# Autodesk Inventor assembly: SHOT_1_002_ShooterAssembly
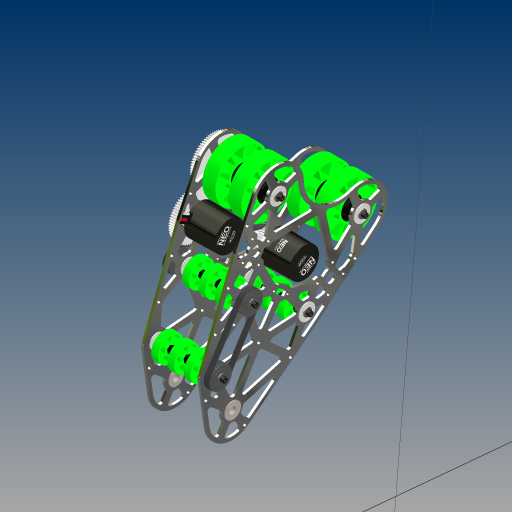
[picture p0: Inventor's stored thumbnail of the model, 512x512]
Saved by Autodesk Inventor 2024.3 (Build 283343000, 343)
## iProperties
Created: 2024-08-07
Part Number: SHOT_1_002_ShooterAssembly
Document SubType Name: Assembly
Designer: Kenji
Mass: 1474.99 g
Surface Area: 3908.93 cm^2
Volume: 710.058 cm^3
Density: 2.07728 g/cm^3
Author: Kenji
## Documents named in this file (27)
- C:\Users\Kenji\Documents\GitHub\1622-2024-Summer-CAD-A-Thon\Shooter\SHOT_1_002_ShooterAssembly.iam
- C:\Users\Kenji\Documents\GitHub\1622-2024-Summer-CAD-A-Thon\Shooter\SHOT_1_001_ShooterPlate.ipt
- C:\Users\Kenji\Documents\GitHub\1622-2024-Summer-CAD-A-Thon\COTS Library\Motion\Wheels\Compliant Wheels\4in compliant wheels\0.500in hex bore\COTS_am-3462_4indiameter_0.500inhexbore_durometer35A_CompliantWheel.ipt
- C:\Users\Kenji\Documents\GitHub\1622-2024-Summer-CAD-A-Thon\COTS Library\Motion\Bearings\COTS_WCP-0783_1.125ODHexBearing.ipt
- C:\Users\Kenji\Documents\GitHub\1622-2024-Summer-CAD-A-Thon\COTS Library\Motion\Bearings\COTS_WCP-0781_0.5ODCircularFlangedBearing.ipt
- C:\Users\Kenji\Documents\GitHub\1622-2024-Summer-CAD-A-Thon\COTS Library\Motors\COTS_REV-21-1650-V1.1_Neo1.1.ipt
- C:\Users\Kenji\Documents\GitHub\1622-2024-Summer-CAD-A-Thon\COTS Library\Motion\Wheels\Compliant Wheels\2in compliant wheels\0.500in hex bore\COTS_am-3462_2indiameter_0.500inhexbore_durometer35A_CompliantWheel.ipt
- C:\Users\Kenji\Documents\GitHub\1622-2024-Summer-CAD-A-Thon\COTS Library\Fasteners\Bolts\Button-Head\10-32\COTS_92949A265_1-2in long Stainless Steel Button Head Screw.ipt
- C:\Users\Kenji\Documents\GitHub\1622-2024-Summer-CAD-A-Thon\COTS Library\Motion\Pulleys\HTD5M\10mm Wide\COTS_HTD5M10mm24T_WCP-0564.ipt
- C:\Users\Kenji\Documents\GitHub\1622-2024-Summer-CAD-A-Thon\COTS Library\Adapters\COTS_REV-21-1879_8mmKeyTo0.5Hex.ipt
- C:\Users\Kenji\Documents\GitHub\1622-2024-Summer-CAD-A-Thon\COTS Library\Motion\Gears\20DP gears\Aluminum\COTS_WCP-0171_66T.ipt
- C:\Users\Kenji\Documents\GitHub\1622-2024-Summer-CAD-A-Thon\Shooter\SHOT_1_004_66TGear-24TPulley.ipt
- C:\Users\Kenji\Documents\GitHub\1622-2024-Summer-CAD-A-Thon\COTS Library\Motion\Gears\20DP gears\Aluminum\COTS_WCP-0717_54T.ipt
- C:\Users\Kenji\Documents\GitHub\1622-2024-Summer-CAD-A-Thon\Shooter\SHOT_1_005_36TGear-24TPulley.ipt
- C:\Users\Kenji\Documents\GitHub\1622-2024-Summer-CAD-A-Thon\Shooter\SHOT_1_014_Belt3.ipt
- C:\Users\Kenji\Documents\GitHub\1622-2024-Summer-CAD-A-Thon\Shooter\SHOT_1_013_Belt2.ipt
- C:\Users\Kenji\Documents\GitHub\1622-2024-Summer-CAD-A-Thon\Shooter\SHOT_1_012_Belt1.ipt
- C:\Users\Kenji\Documents\GitHub\1622-2024-Summer-CAD-A-Thon\Shooter\SHOT_1_010_Spacer1.ipt
- C:\Users\Kenji\Documents\GitHub\1622-2024-Summer-CAD-A-Thon\Shooter\SHOT_1_011_Spacer2.ipt
- C:\Users\Kenji\Documents\GitHub\1622-2024-Summer-CAD-A-Thon\Shooter\SHOT_1_006_HexShaft1.ipt
- C:\Users\Kenji\Documents\GitHub\1622-2024-Summer-CAD-A-Thon\Shooter\SHOT_1_007_HexShaft2.ipt
- C:\Users\Kenji\Documents\GitHub\1622-2024-Summer-CAD-A-Thon\Shooter\SHOT_1_008_HexShaft3.ipt
- C:\Users\Kenji\Documents\GitHub\1622-2024-Summer-CAD-A-Thon\Shooter\SHOT_1_009_HexShaft4.ipt
- C:\Users\Kenji\Documents\GitHub\1622-2024-Summer-CAD-A-Thon\COTS Library\Fasteners\Bolts\Socket-Head\0.25-20\COTS_91251A539_Black-Oxide Alloy Steel Socket Head Screw (1).ipt
- C:\Users\Kenji\Documents\GitHub\1622-2024-Summer-CAD-A-Thon\COTS Library\Fasteners\Washers\COTS_90107A029_316 Stainless Steel Washer.ipt
- C:\Users\Kenji\Documents\GitHub\1622-2024-Summer-CAD-A-Thon\COTS Library\Fasteners\Bolts\Button-Head\10-32\COTS_92949A267_18-8 Stainless Steel Button Head Hex Drive Screw (1).ipt
- C:\Users\Kenji\Documents\GitHub\1622-2024-Summer-CAD-A-Thon\COTS Library\Fasteners\Washers\COTS_91860A047_Size10Washer.ipt
## Components (85 placed, 26 different names)
1. SHOT_1_001_ShooterPlate:1 — Mate:140, Mate:141, Mate:142, Mate:143, Mate:144, Mate:148, Mate:150, Mate:151, Mate:152, Mate:160, Mate:161, Mate:163, Mate:164, Mate:165, Mate:166, Mate:167, Mate:168, Mate:169, Mate:170, Mate:171, Mate:172, Mate:270, Mate:271, Mate:280, Mate:281, Mate:282, Mate:283, Mate:284, Mate:285, Mate:286, Mate:287, Mate:288, Mate:289, Mate:290, Mate:294, Mate:304, Mate:305
2. SHOT_1_001_ShooterPlate:2 — Mate:140, Mate:141, Mate:147, Mate:149, Mate:156, Mate:158, Mate:159, Mate:272, Mate:273, Mate:304, Mate:311
3. COTS_WCP-0783_1.125ODHexBearing:1 — Mate:139, Flush:5, Mate:156, Mate:246
4. COTS_WCP-0783_1.125ODHexBearing:2 — Mate:146, Mate:147, Mate:149, Mate:299
5. COTS_WCP-0783_1.125ODHexBearing:3 — Mate:36, Mate:102, Flush:5, Mate:251
6. COTS_WCP-0783_1.125ODHexBearing:5 — Mate:244, Mate:270, Mate:271, Mate:274, Mate:275
7. COTS_WCP-0783_1.125ODHexBearing:9 — Mate:102, Flush:4, Mate:150, Mate:152, Mate:186, Mate:187
8. COTS_WCP-0783_1.125ODHexBearing:10 — Mate:31, Mate:104, Flush:4, Mate:151, Mate:188, Mate:213
9. COTS_WCP-0783_1.125ODHexBearing:11 — Mate:49, Mate:52, Mate:143, Mate:144, Flush:17
10. COTS_WCP-0783_1.125ODHexBearing:12 — Mate:272, Mate:273, Mate:278
11. COTS_WCP-0781_0.5ODCircularFlangedBearing:1 — Mate:138, Mate:158, Mate:159
12. COTS_WCP-0781_0.5ODCircularFlangedBearing:2 — Mate:138, Mate:160
13. COTS_REV-21-1650-V1.1_Neo1.1:1 — Mate:133, Mate:161, Mate:163, Mate:185, Mate:256, Mate:260, Mate:261, Mate:266
14. COTS_92949A265_1-2in long Stainless Steel Button Head Screw:1 — Mate:165, Mate:168, Mate:185
15. COTS_92949A265_1-2in long Stainless Steel Button Head Screw:2 — Mate:167, Mate:170
16. COTS_92949A265_1-2in long Stainless Steel Button Head Screw:3 — Mate:166, Mate:169
17. COTS_92949A265_1-2in long Stainless Steel Button Head Screw:4 — Mate:164, Mate:171
18. COTS_WCP-0783_1.125ODHexBearing:13 — Mate:148, Mate:297, Mate:305, Mate:306
19. COTS_WCP-0783_1.125ODHexBearing:14 — Mate:134, Mate:308, Mate:311, Mate:315
20. COTS_REV-21-1650-V1.1_Neo1.1:2 — Mate:280, Mate:281, Mate:282, Mate:291, Mate:292, Mate:293, Mate:295
21. COTS_REV-21-1879_8mmKeyTo0.5Hex:1 — Mate:291, Mate:292
22. COTS_92949A265_1-2in long Stainless Steel Button Head Screw:5 — Mate:285, Mate:288
23. COTS_92949A265_1-2in long Stainless Steel Button Head Screw:6 — Mate:286, Mate:290
24. COTS_92949A265_1-2in long Stainless Steel Button Head Screw:7 — Mate:283, Mate:287
25. COTS_92949A265_1-2in long Stainless Steel Button Head Screw:8 — Mate:284, Mate:289
26. SHOT_1_004_66TGear-24TPulley:1 — Mate:133, Mate:172, Flush:6, Mate:198, Mate:257
27. COTS_WCP-0171_66T:1 — Mate:186, Mate:187, Mate:301, Flush:15
28. COTS_HTD5M10mm24T_WCP-0564:1 — Mate:188, Flush:6, Mate:199, Mate:200, Mate:207, Flush:9, Mate:214, Mate:240
29. COTS_WCP-0717_54T:1 — Mate:274, Mate:275, Mate:276, Flush:13, Mate:329, Mate:330
30. SHOT_1_005_36TGear-24TPulley:1 — Mate:293, Mate:294, Mate:296, Flush:16, Mate:318, Mate:319
31. COTS_HTD5M10mm24T_WCP-0564:2 — Mate:298, Flush:14, Mate:299, Mate:320, Mate:323
32. COTS_HTD5M10mm24T_WCP-0564:3 — Mate:300, Flush:16, Mate:307, Mate:317, Mate:326
33. COTS_HTD5M10mm24T_WCP-0564:4 — Mate:255, Mate:314, Mate:315, Mate:321
34. SHOT_1_014_Belt3:1 — Mate:255, Mate:320, Mate:321
35. SHOT_1_013_Belt2:1 — Mate:317, Mate:318, Mate:319
36. SHOT_1_012_Belt1:1 — Mate:198, Mate:199, Mate:200
37. SHOT_1_010_Spacer1:1 — Mate:213, Mate:214
38. SHOT_1_010_Spacer1:2 — Mate:306, Mate:307
39. SHOT_1_006_HexShaft1:1 — Mate:235, Mate:301, Flush:15, Mate:302, Mate:303
40. SHOT_1_007_HexShaft2:1 — Mate:207, Flush:9, Mate:238, Mate:245
41. SHOT_1_008_HexShaft3:1 — Mate:297, Mate:298, Flush:14, Mate:300, Mate:322, Mate:325
42. SHOT_1_009_HexShaft4:1 — Mate:237, Mate:248, Mate:308, Flush:17, Mate:310, Mate:312
43. SHOT_1_006_HexShaft1:2 — Mate:239, Mate:249, Mate:276, Flush:13, Mate:277
44. COTS_91251A539_Black-Oxide Alloy Steel Socket Head Screw (1):1 — Mate:219, Mate:233, Mate:239
45. COTS_91251A539_Black-Oxide Alloy Steel Socket Head Screw (1):2 — Mate:220, Mate:230, Mate:238
46. COTS_91251A539_Black-Oxide Alloy Steel Socket Head Screw (1):3 — Mate:222, Mate:229, Mate:249
47. COTS_91251A539_Black-Oxide Alloy Steel Socket Head Screw (1):4 — Mate:217, Mate:232, Mate:303
48. COTS_91251A539_Black-Oxide Alloy Steel Socket Head Screw (1):5 — Mate:218, Mate:234, Mate:235
49. COTS_91251A539_Black-Oxide Alloy Steel Socket Head Screw (1):6 — Mate:316, Mate:322, Mate:324
50. COTS_91251A539_Black-Oxide Alloy Steel Socket Head Screw (1):7 — Mate:224, Mate:237, Mate:309
51. COTS_91251A539_Black-Oxide Alloy Steel Socket Head Screw (1):8 — Mate:223, Mate:227, Mate:325
52. COTS_91251A539_Black-Oxide Alloy Steel Socket Head Screw (1):9 — Mate:216, Mate:248, Mate:313, Mate:314
53. COTS_91251A539_Black-Oxide Alloy Steel Socket Head Screw (1):10 — Mate:215, Mate:231, Mate:245
54. COTS_90107A029_316 Stainless Steel Washer:1 — Mate:218, Mate:234, Mate:302
55. COTS_90107A029_316 Stainless Steel Washer:2 — Mate:220, Mate:230, Mate:240
56. COTS_90107A029_316 Stainless Steel Washer:3 — Mate:316, Mate:323, Mate:324
57. COTS_90107A029_316 Stainless Steel Washer:4 — Mate:219, Mate:233, Mate:244
58. COTS_90107A029_316 Stainless Steel Washer:5 — Mate:222, Mate:229, Mate:278
59. COTS_90107A029_316 Stainless Steel Washer:6 — Mate:223, Mate:227, Mate:326
60. COTS_90107A029_316 Stainless Steel Washer:7 — Mate:224, Mate:309, Mate:310
61. COTS_90107A029_316 Stainless Steel Washer:8 — Mate:217, Mate:232, Mate:251
62. COTS_90107A029_316 Stainless Steel Washer:9 — Mate:215, Mate:231, Mate:246
63. COTS_90107A029_316 Stainless Steel Washer:10 — Mate:216, Mate:312, Mate:313
64. SHOT_1_011_Spacer2:1 — Mate:256, Mate:257, Mate:267
65. SHOT_1_011_Spacer2:2 — Mate:269, Mate:279, Mate:296
66. COTS_REV-21-1879_8mmKeyTo0.5Hex:2 — Mate:260, Mate:261
67. COTS_92949A267_18-8 Stainless Steel Button Head Hex Drive Screw (1):1 — Mate:263, Mate:265, Mate:266
68. COTS_92949A267_18-8 Stainless Steel Button Head Hex Drive Screw (1):2 — Mate:262, Mate:264, Mate:279, Mate:295
69. COTS_91860A047_Size10Washer:1 — Mate:262, Mate:264, Mate:269
70. COTS_91860A047_Size10Washer:2 — Mate:263, Mate:265, Mate:267
71. COTS_90107A029_316 Stainless Steel Washer:11 — Mate:327, Mate:328, Mate:329, Mate:330
72. COTS_91251A539_Black-Oxide Alloy Steel Socket Head Screw (1):11 — Mate:327, Mate:328
73. COTS_am-3462_4indiameter_0.500inhexbore_durometer35A_CompliantWheel:4 — Mate:36, Flush:3
74. COTS_am-3462_4indiameter_0.500inhexbore_durometer35A_CompliantWheel:1 — Mate:31, Flush:3, Mate:104
75. COTS_am-3462_4indiameter_0.500inhexbore_durometer35A_CompliantWheel:5
76. COTS_am-3462_4indiameter_0.500inhexbore_durometer35A_CompliantWheel:6 — Mate:139
77. COTS_am-3462_2indiameter_0.500inhexbore_durometer35A_CompliantWheel:2 — Mate:49, Flush:1, Mate:52
78. COTS_am-3462_2indiameter_0.500inhexbore_durometer35A_CompliantWheel:6 — Flush:2
79. COTS_am-3462_2indiameter_0.500inhexbore_durometer35A_CompliantWheel:1 — Flush:1, Flush:2
80. COTS_am-3462_2indiameter_0.500inhexbore_durometer35A_CompliantWheel:7 — Mate:142
81. COTS_am-3462_2indiameter_0.500inhexbore_durometer35A_CompliantWheel:8
82. COTS_am-3462_2indiameter_0.500inhexbore_durometer35A_CompliantWheel:9
83. COTS_am-3462_2indiameter_0.500inhexbore_durometer35A_CompliantWheel:10 — Mate:134
84. COTS_am-3462_2indiameter_0.500inhexbore_durometer35A_CompliantWheel:11 — Mate:146
85. COTS_am-3462_2indiameter_0.500inhexbore_durometer35A_CompliantWheel:12 — Mate:277
## Component patterns: (2 elements, first: COTS_am-3462_4indiameter_0.500inhexbore_durometer35A_CompliantWheel:4 + COTS_am-3462_4indiameter_0.500inhexbore_durometer35A_CompliantWheel:1), (3 elements, first: COTS_am-3462_2indiameter_0.500inhexbore_durometer35A_CompliantWheel:2 + COTS_am-3462_2indiameter_0.500inhexbore_durometer35A_CompliantWheel:6 + COTS_am-3462_2indiameter_0.500inhexbore_durometer35A_CompliantWheel:1)
## Relationships (159: Mate 147, Flush 12)
- Mate:31: COTS_WCP-0783_1.125ODHexBearing:10 ↔ COTS_am-3462_4indiameter_0.500inhexbore_durometer35A_CompliantWheel:1
- Mate:36: COTS_WCP-0783_1.125ODHexBearing:3 ↔ COTS_am-3462_4indiameter_0.500inhexbore_durometer35A_CompliantWheel:4
- Mate:49: COTS_WCP-0783_1.125ODHexBearing:11 ↔ COTS_am-3462_2indiameter_0.500inhexbore_durometer35A_CompliantWheel:2
- Flush:1: COTS_am-3462_2indiameter_0.500inhexbore_durometer35A_CompliantWheel:2 ↔ COTS_am-3462_2indiameter_0.500inhexbore_durometer35A_CompliantWheel:1
- Flush:2: COTS_am-3462_2indiameter_0.500inhexbore_durometer35A_CompliantWheel:6 ↔ COTS_am-3462_2indiameter_0.500inhexbore_durometer35A_CompliantWheel:1
- Mate:52 (12.7 mm): COTS_WCP-0783_1.125ODHexBearing:11 ↔ COTS_am-3462_2indiameter_0.500inhexbore_durometer35A_CompliantWheel:2
- Mate:102: COTS_WCP-0783_1.125ODHexBearing:3 ↔ COTS_WCP-0783_1.125ODHexBearing:9
- Flush:3: COTS_am-3462_4indiameter_0.500inhexbore_durometer35A_CompliantWheel:4 ↔ COTS_am-3462_4indiameter_0.500inhexbore_durometer35A_CompliantWheel:1
- Mate:104 (12.7 mm): COTS_WCP-0783_1.125ODHexBearing:10 ↔ COTS_am-3462_4indiameter_0.500inhexbore_durometer35A_CompliantWheel:1
- Mate:133: COTS_REV-21-1650-V1.1_Neo1.1:1 ↔ SHOT_1_004_66TGear-24TPulley:1
- Mate:134: COTS_WCP-0783_1.125ODHexBearing:14 ↔ COTS_am-3462_2indiameter_0.500inhexbore_durometer35A_CompliantWheel:10
- Mate:138: COTS_WCP-0781_0.5ODCircularFlangedBearing:1 ↔ COTS_WCP-0781_0.5ODCircularFlangedBearing:2
- Mate:139: COTS_WCP-0783_1.125ODHexBearing:1 ↔ COTS_am-3462_4indiameter_0.500inhexbore_durometer35A_CompliantWheel:6
- Flush:4: COTS_WCP-0783_1.125ODHexBearing:9 ↔ COTS_WCP-0783_1.125ODHexBearing:10
- Flush:5: COTS_WCP-0783_1.125ODHexBearing:1 ↔ COTS_WCP-0783_1.125ODHexBearing:3
- Mate:140: SHOT_1_001_ShooterPlate:1 ↔ SHOT_1_001_ShooterPlate:2
- Mate:141: SHOT_1_001_ShooterPlate:1 ↔ SHOT_1_001_ShooterPlate:2
- Mate:142: SHOT_1_001_ShooterPlate:1 ↔ COTS_am-3462_2indiameter_0.500inhexbore_durometer35A_CompliantWheel:7
- Mate:143: SHOT_1_001_ShooterPlate:1 ↔ COTS_WCP-0783_1.125ODHexBearing:11
- Mate:144: SHOT_1_001_ShooterPlate:1 ↔ COTS_WCP-0783_1.125ODHexBearing:11
- Mate:146: COTS_WCP-0783_1.125ODHexBearing:2 ↔ COTS_am-3462_2indiameter_0.500inhexbore_durometer35A_CompliantWheel:11
- Mate:147: SHOT_1_001_ShooterPlate:2 ↔ COTS_WCP-0783_1.125ODHexBearing:2
- Mate:148: SHOT_1_001_ShooterPlate:1 ↔ COTS_WCP-0783_1.125ODHexBearing:13
- Mate:149: SHOT_1_001_ShooterPlate:2 ↔ COTS_WCP-0783_1.125ODHexBearing:2
- Mate:150: SHOT_1_001_ShooterPlate:1 ↔ COTS_WCP-0783_1.125ODHexBearing:9
- Mate:151: SHOT_1_001_ShooterPlate:1 ↔ COTS_WCP-0783_1.125ODHexBearing:10
- Mate:152: SHOT_1_001_ShooterPlate:1 ↔ COTS_WCP-0783_1.125ODHexBearing:9
- Mate:156: SHOT_1_001_ShooterPlate:2 ↔ COTS_WCP-0783_1.125ODHexBearing:1
- Mate:158: SHOT_1_001_ShooterPlate:2 ↔ COTS_WCP-0781_0.5ODCircularFlangedBearing:1
- Mate:159: SHOT_1_001_ShooterPlate:2 ↔ COTS_WCP-0781_0.5ODCircularFlangedBearing:1
- Mate:160: SHOT_1_001_ShooterPlate:1 ↔ COTS_WCP-0781_0.5ODCircularFlangedBearing:2
- Mate:161: SHOT_1_001_ShooterPlate:1 ↔ COTS_REV-21-1650-V1.1_Neo1.1:1
- Mate:163: SHOT_1_001_ShooterPlate:1 ↔ COTS_REV-21-1650-V1.1_Neo1.1:1
- Mate:164: SHOT_1_001_ShooterPlate:1 ↔ COTS_92949A265_1-2in long Stainless Steel Button Head Screw:4
- Mate:165: SHOT_1_001_ShooterPlate:1 ↔ COTS_92949A265_1-2in long Stainless Steel Button Head Screw:1
- Mate:166: SHOT_1_001_ShooterPlate:1 ↔ COTS_92949A265_1-2in long Stainless Steel Button Head Screw:3
- Mate:167: SHOT_1_001_ShooterPlate:1 ↔ COTS_92949A265_1-2in long Stainless Steel Button Head Screw:2
- Mate:168: SHOT_1_001_ShooterPlate:1 ↔ COTS_92949A265_1-2in long Stainless Steel Button Head Screw:1
- Mate:169: SHOT_1_001_ShooterPlate:1 ↔ COTS_92949A265_1-2in long Stainless Steel Button Head Screw:3
- Mate:170: SHOT_1_001_ShooterPlate:1 ↔ COTS_92949A265_1-2in long Stainless Steel Button Head Screw:2
- Mate:171: SHOT_1_001_ShooterPlate:1 ↔ COTS_92949A265_1-2in long Stainless Steel Button Head Screw:4
- Mate:172: SHOT_1_001_ShooterPlate:1 ↔ SHOT_1_004_66TGear-24TPulley:1
- Mate:185: COTS_REV-21-1650-V1.1_Neo1.1:1 ↔ COTS_92949A265_1-2in long Stainless Steel Button Head Screw:1
- Mate:186: COTS_WCP-0783_1.125ODHexBearing:9 ↔ COTS_WCP-0171_66T:1
- Mate:187: COTS_WCP-0783_1.125ODHexBearing:9 ↔ COTS_WCP-0171_66T:1
- Mate:188: COTS_WCP-0783_1.125ODHexBearing:10 ↔ COTS_HTD5M10mm24T_WCP-0564:1
- Flush:6: SHOT_1_004_66TGear-24TPulley:1 ↔ COTS_HTD5M10mm24T_WCP-0564:1
- Mate:198: SHOT_1_004_66TGear-24TPulley:1 ↔ SHOT_1_012_Belt1:1
- Mate:199: COTS_HTD5M10mm24T_WCP-0564:1 ↔ SHOT_1_012_Belt1:1
- Mate:200: COTS_HTD5M10mm24T_WCP-0564:1 ↔ SHOT_1_012_Belt1:1
- Mate:207: COTS_HTD5M10mm24T_WCP-0564:1 ↔ SHOT_1_007_HexShaft2:1
- Flush:9: COTS_HTD5M10mm24T_WCP-0564:1 ↔ SHOT_1_007_HexShaft2:1
- Mate:213: COTS_WCP-0783_1.125ODHexBearing:10 ↔ SHOT_1_010_Spacer1:1
- Mate:214: COTS_HTD5M10mm24T_WCP-0564:1 ↔ SHOT_1_010_Spacer1:1
- Mate:215: COTS_91251A539_Black-Oxide Alloy Steel Socket Head Screw (1):10 ↔ COTS_90107A029_316 Stainless Steel Washer:9
- Mate:216: COTS_91251A539_Black-Oxide Alloy Steel Socket Head Screw (1):9 ↔ COTS_90107A029_316 Stainless Steel Washer:10
- Mate:217: COTS_91251A539_Black-Oxide Alloy Steel Socket Head Screw (1):4 ↔ COTS_90107A029_316 Stainless Steel Washer:8
- Mate:218: COTS_91251A539_Black-Oxide Alloy Steel Socket Head Screw (1):5 ↔ COTS_90107A029_316 Stainless Steel Washer:1
- Mate:219: COTS_91251A539_Black-Oxide Alloy Steel Socket Head Screw (1):1 ↔ COTS_90107A029_316 Stainless Steel Washer:4
- Mate:220: COTS_91251A539_Black-Oxide Alloy Steel Socket Head Screw (1):2 ↔ COTS_90107A029_316 Stainless Steel Washer:2
- Mate:222: COTS_91251A539_Black-Oxide Alloy Steel Socket Head Screw (1):3 ↔ COTS_90107A029_316 Stainless Steel Washer:5
- Mate:223: COTS_91251A539_Black-Oxide Alloy Steel Socket Head Screw (1):8 ↔ COTS_90107A029_316 Stainless Steel Washer:6
- Mate:224: COTS_91251A539_Black-Oxide Alloy Steel Socket Head Screw (1):7 ↔ COTS_90107A029_316 Stainless Steel Washer:7
- Mate:227: COTS_91251A539_Black-Oxide Alloy Steel Socket Head Screw (1):8 ↔ COTS_90107A029_316 Stainless Steel Washer:6
- Mate:229: COTS_91251A539_Black-Oxide Alloy Steel Socket Head Screw (1):3 ↔ COTS_90107A029_316 Stainless Steel Washer:5
- Mate:230: COTS_91251A539_Black-Oxide Alloy Steel Socket Head Screw (1):2 ↔ COTS_90107A029_316 Stainless Steel Washer:2
- Mate:231: COTS_91251A539_Black-Oxide Alloy Steel Socket Head Screw (1):10 ↔ COTS_90107A029_316 Stainless Steel Washer:9
- Mate:232: COTS_91251A539_Black-Oxide Alloy Steel Socket Head Screw (1):4 ↔ COTS_90107A029_316 Stainless Steel Washer:8
- Mate:233: COTS_91251A539_Black-Oxide Alloy Steel Socket Head Screw (1):1 ↔ COTS_90107A029_316 Stainless Steel Washer:4
- Mate:234: COTS_91251A539_Black-Oxide Alloy Steel Socket Head Screw (1):5 ↔ COTS_90107A029_316 Stainless Steel Washer:1
- Mate:235: SHOT_1_006_HexShaft1:1 ↔ COTS_91251A539_Black-Oxide Alloy Steel Socket Head Screw (1):5
- Mate:237: SHOT_1_009_HexShaft4:1 ↔ COTS_91251A539_Black-Oxide Alloy Steel Socket Head Screw (1):7
- Mate:238: SHOT_1_007_HexShaft2:1 ↔ COTS_91251A539_Black-Oxide Alloy Steel Socket Head Screw (1):2
- Mate:239: SHOT_1_006_HexShaft1:2 ↔ COTS_91251A539_Black-Oxide Alloy Steel Socket Head Screw (1):1
- Mate:240: COTS_HTD5M10mm24T_WCP-0564:1 ↔ COTS_90107A029_316 Stainless Steel Washer:2
- Mate:244: COTS_WCP-0783_1.125ODHexBearing:5 ↔ COTS_90107A029_316 Stainless Steel Washer:4
- Mate:245: SHOT_1_007_HexShaft2:1 ↔ COTS_91251A539_Black-Oxide Alloy Steel Socket Head Screw (1):10
- Mate:246: COTS_WCP-0783_1.125ODHexBearing:1 ↔ COTS_90107A029_316 Stainless Steel Washer:9
- Mate:248: SHOT_1_009_HexShaft4:1 ↔ COTS_91251A539_Black-Oxide Alloy Steel Socket Head Screw (1):9
- Mate:249: SHOT_1_006_HexShaft1:2 ↔ COTS_91251A539_Black-Oxide Alloy Steel Socket Head Screw (1):3
- Mate:251: COTS_WCP-0783_1.125ODHexBearing:3 ↔ COTS_90107A029_316 Stainless Steel Washer:8
- Mate:255: COTS_HTD5M10mm24T_WCP-0564:4 ↔ SHOT_1_014_Belt3:1
- Mate:256: COTS_REV-21-1650-V1.1_Neo1.1:1 ↔ SHOT_1_011_Spacer2:1
- Mate:257: SHOT_1_004_66TGear-24TPulley:1 ↔ SHOT_1_011_Spacer2:1
- Mate:260: COTS_REV-21-1650-V1.1_Neo1.1:1 ↔ COTS_REV-21-1879_8mmKeyTo0.5Hex:2
- Mate:261: COTS_REV-21-1650-V1.1_Neo1.1:1 ↔ COTS_REV-21-1879_8mmKeyTo0.5Hex:2
- Mate:262: COTS_92949A267_18-8 Stainless Steel Button Head Hex Drive Screw (1):2 ↔ COTS_91860A047_Size10Washer:1
- Mate:263: COTS_92949A267_18-8 Stainless Steel Button Head Hex Drive Screw (1):1 ↔ COTS_91860A047_Size10Washer:2
- Mate:264: COTS_92949A267_18-8 Stainless Steel Button Head Hex Drive Screw (1):2 ↔ COTS_91860A047_Size10Washer:1
- Mate:265: COTS_92949A267_18-8 Stainless Steel Button Head Hex Drive Screw (1):1 ↔ COTS_91860A047_Size10Washer:2
- Mate:266: COTS_REV-21-1650-V1.1_Neo1.1:1 ↔ COTS_92949A267_18-8 Stainless Steel Button Head Hex Drive Screw (1):1
- Mate:267: SHOT_1_011_Spacer2:1 ↔ COTS_91860A047_Size10Washer:2
- Mate:269: SHOT_1_011_Spacer2:2 ↔ COTS_91860A047_Size10Washer:1
- Mate:270: SHOT_1_001_ShooterPlate:1 ↔ COTS_WCP-0783_1.125ODHexBearing:5
- Mate:271: SHOT_1_001_ShooterPlate:1 ↔ COTS_WCP-0783_1.125ODHexBearing:5
- Mate:272: SHOT_1_001_ShooterPlate:2 ↔ COTS_WCP-0783_1.125ODHexBearing:12
- Mate:273: SHOT_1_001_ShooterPlate:2 ↔ COTS_WCP-0783_1.125ODHexBearing:12
- Mate:274: COTS_WCP-0783_1.125ODHexBearing:5 ↔ COTS_WCP-0717_54T:1
- Mate:275: COTS_WCP-0783_1.125ODHexBearing:5 ↔ COTS_WCP-0717_54T:1
- Mate:276: COTS_WCP-0717_54T:1 ↔ SHOT_1_006_HexShaft1:2
- Flush:13: COTS_WCP-0717_54T:1 ↔ SHOT_1_006_HexShaft1:2
- Mate:277: SHOT_1_006_HexShaft1:2 ↔ COTS_am-3462_2indiameter_0.500inhexbore_durometer35A_CompliantWheel:12
- Mate:278: COTS_WCP-0783_1.125ODHexBearing:12 ↔ COTS_90107A029_316 Stainless Steel Washer:5
- Mate:279: SHOT_1_011_Spacer2:2 ↔ COTS_92949A267_18-8 Stainless Steel Button Head Hex Drive Screw (1):2
- Mate:280: SHOT_1_001_ShooterPlate:1 ↔ COTS_REV-21-1650-V1.1_Neo1.1:2
- Mate:281: SHOT_1_001_ShooterPlate:1 ↔ COTS_REV-21-1650-V1.1_Neo1.1:2
- Mate:282: SHOT_1_001_ShooterPlate:1 ↔ COTS_REV-21-1650-V1.1_Neo1.1:2
- Mate:283: SHOT_1_001_ShooterPlate:1 ↔ COTS_92949A265_1-2in long Stainless Steel Button Head Screw:7
- Mate:284: SHOT_1_001_ShooterPlate:1 ↔ COTS_92949A265_1-2in long Stainless Steel Button Head Screw:8
- Mate:285: SHOT_1_001_ShooterPlate:1 ↔ COTS_92949A265_1-2in long Stainless Steel Button Head Screw:5
- Mate:286: SHOT_1_001_ShooterPlate:1 ↔ COTS_92949A265_1-2in long Stainless Steel Button Head Screw:6
- Mate:287: SHOT_1_001_ShooterPlate:1 ↔ COTS_92949A265_1-2in long Stainless Steel Button Head Screw:7
- Mate:288: SHOT_1_001_ShooterPlate:1 ↔ COTS_92949A265_1-2in long Stainless Steel Button Head Screw:5
- Mate:289: SHOT_1_001_ShooterPlate:1 ↔ COTS_92949A265_1-2in long Stainless Steel Button Head Screw:8
- Mate:290: SHOT_1_001_ShooterPlate:1 ↔ COTS_92949A265_1-2in long Stainless Steel Button Head Screw:6
- Mate:291: COTS_REV-21-1650-V1.1_Neo1.1:2 ↔ COTS_REV-21-1879_8mmKeyTo0.5Hex:1
- Mate:292: COTS_REV-21-1650-V1.1_Neo1.1:2 ↔ COTS_REV-21-1879_8mmKeyTo0.5Hex:1
- Mate:293: COTS_REV-21-1650-V1.1_Neo1.1:2 ↔ SHOT_1_005_36TGear-24TPulley:1
- Mate:294: SHOT_1_001_ShooterPlate:1 ↔ SHOT_1_005_36TGear-24TPulley:1
- Mate:295: COTS_REV-21-1650-V1.1_Neo1.1:2 ↔ COTS_92949A267_18-8 Stainless Steel Button Head Hex Drive Screw (1):2
- Mate:296: SHOT_1_005_36TGear-24TPulley:1 ↔ SHOT_1_011_Spacer2:2
- Mate:297: COTS_WCP-0783_1.125ODHexBearing:13 ↔ SHOT_1_008_HexShaft3:1
- Mate:298: COTS_HTD5M10mm24T_WCP-0564:2 ↔ SHOT_1_008_HexShaft3:1
- Flush:14: COTS_HTD5M10mm24T_WCP-0564:2 ↔ SHOT_1_008_HexShaft3:1
- Mate:299: COTS_WCP-0783_1.125ODHexBearing:2 ↔ COTS_HTD5M10mm24T_WCP-0564:2
- Mate:300: COTS_HTD5M10mm24T_WCP-0564:3 ↔ SHOT_1_008_HexShaft3:1
- Mate:301: COTS_WCP-0171_66T:1 ↔ SHOT_1_006_HexShaft1:1
- Flush:15: COTS_WCP-0171_66T:1 ↔ SHOT_1_006_HexShaft1:1
- Mate:302: SHOT_1_006_HexShaft1:1 ↔ COTS_90107A029_316 Stainless Steel Washer:1
- Mate:303: SHOT_1_006_HexShaft1:1 ↔ COTS_91251A539_Black-Oxide Alloy Steel Socket Head Screw (1):4
- Mate:304 (104.775 mm): SHOT_1_001_ShooterPlate:1 ↔ SHOT_1_001_ShooterPlate:2
- Mate:305: SHOT_1_001_ShooterPlate:1 ↔ COTS_WCP-0783_1.125ODHexBearing:13
- Flush:16: SHOT_1_005_36TGear-24TPulley:1 ↔ COTS_HTD5M10mm24T_WCP-0564:3
- Mate:306: COTS_WCP-0783_1.125ODHexBearing:13 ↔ SHOT_1_010_Spacer1:2
- Mate:307: COTS_HTD5M10mm24T_WCP-0564:3 ↔ SHOT_1_010_Spacer1:2
- Mate:308: COTS_WCP-0783_1.125ODHexBearing:14 ↔ SHOT_1_009_HexShaft4:1
- Flush:17: COTS_WCP-0783_1.125ODHexBearing:11 ↔ SHOT_1_009_HexShaft4:1
- Mate:309: COTS_91251A539_Black-Oxide Alloy Steel Socket Head Screw (1):7 ↔ COTS_90107A029_316 Stainless Steel Washer:7
- Mate:310: SHOT_1_009_HexShaft4:1 ↔ COTS_90107A029_316 Stainless Steel Washer:7
- Mate:311: SHOT_1_001_ShooterPlate:2 ↔ COTS_WCP-0783_1.125ODHexBearing:14
- Mate:312: SHOT_1_009_HexShaft4:1 ↔ COTS_90107A029_316 Stainless Steel Washer:10
- Mate:313: COTS_91251A539_Black-Oxide Alloy Steel Socket Head Screw (1):9 ↔ COTS_90107A029_316 Stainless Steel Washer:10
- Mate:314: COTS_HTD5M10mm24T_WCP-0564:4 ↔ COTS_91251A539_Black-Oxide Alloy Steel Socket Head Screw (1):9
- Mate:315: COTS_WCP-0783_1.125ODHexBearing:14 ↔ COTS_HTD5M10mm24T_WCP-0564:4
- Mate:316: COTS_91251A539_Black-Oxide Alloy Steel Socket Head Screw (1):6 ↔ COTS_90107A029_316 Stainless Steel Washer:3
- Mate:317: COTS_HTD5M10mm24T_WCP-0564:3 ↔ SHOT_1_013_Belt2:1
- Mate:318: SHOT_1_005_36TGear-24TPulley:1 ↔ SHOT_1_013_Belt2:1
- Mate:319: SHOT_1_005_36TGear-24TPulley:1 ↔ SHOT_1_013_Belt2:1
- Mate:320: COTS_HTD5M10mm24T_WCP-0564:2 ↔ SHOT_1_014_Belt3:1
- Mate:321: COTS_HTD5M10mm24T_WCP-0564:4 ↔ SHOT_1_014_Belt3:1
- Mate:322: SHOT_1_008_HexShaft3:1 ↔ COTS_91251A539_Black-Oxide Alloy Steel Socket Head Screw (1):6
- Mate:323: COTS_HTD5M10mm24T_WCP-0564:2 ↔ COTS_90107A029_316 Stainless Steel Washer:3
- Mate:324: COTS_91251A539_Black-Oxide Alloy Steel Socket Head Screw (1):6 ↔ COTS_90107A029_316 Stainless Steel Washer:3
- Mate:325: SHOT_1_008_HexShaft3:1 ↔ COTS_91251A539_Black-Oxide Alloy Steel Socket Head Screw (1):8
- Mate:326: COTS_HTD5M10mm24T_WCP-0564:3 ↔ COTS_90107A029_316 Stainless Steel Washer:6
- Mate:327: COTS_90107A029_316 Stainless Steel Washer:11 ↔ COTS_91251A539_Black-Oxide Alloy Steel Socket Head Screw (1):11
- Mate:328: COTS_90107A029_316 Stainless Steel Washer:11 ↔ COTS_91251A539_Black-Oxide Alloy Steel Socket Head Screw (1):11
- Mate:329: COTS_WCP-0717_54T:1 ↔ COTS_90107A029_316 Stainless Steel Washer:11
- Mate:330: COTS_WCP-0717_54T:1 ↔ COTS_90107A029_316 Stainless Steel Washer:11
